# Autodesk Inventor assembly: Assembly1
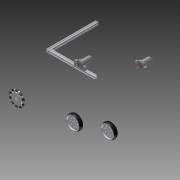
[picture p0: Inventor's stored thumbnail of the model, 180x180]
Saved by Autodesk Inventor 2013 (Build 170138000, 138)
## iProperties
Created: 2013-11-11
Part Number: Assembly1
Document SubType Name: Assembly
Designer: cobrooks
Author: cobrooks
## Documents named in this file (7)
- C:\Users\cobrooks\Documents\GitHub\2013-2014_BlockParty\CAD\Drive\WIMP_mk2\Assembly1.iam
- C:\Users\cobrooks\Documents\GitHub\2013-2014_BlockParty\CAD\COTSParts\Tetrix\Tetrix wheel 4 in.ipt
- C:\Users\cobrooks\Documents\GitHub\2013-2014_BlockParty\CAD\Drive\WIMP_mk2\DriveSide.ipt
- C:\Users\cobrooks\Documents\GitHub\2013-2014_BlockParty\CAD\COTSParts\Tetrix\Tetrix motor mount.ipt
- C:\Users\cobrooks\Documents\GitHub\2013-2014_BlockParty\CAD\Drive\WIMP_mk2\DriveBack.ipt
- C:\Users\cobrooks\Documents\GitHub\2013-2014_BlockParty\CAD\COTSParts\Tetrix\Tetrix motor.ipt
- C:\Users\cobrooks\Documents\GitHub\2013-2014_BlockParty\CAD\Drive\Final Drive Complete\Tetrix Wheel 4 in omni.ipt
## Components (9 placed, 6 different names)
1. Tetrix wheel 4 in:1 — Flush:1, Mate:1
2. Tetrix wheel 4 in:3 — Flush:1, Mate:4
3. DriveSide:1 — Mate:4, Mate:5, Flush:2, Flush:3, Flush:4, Mate:6, Flush:5
4. Tetrix motor mount:1 — Insert:1
5. Tetrix motor mount:2 — Insert:2, Flush:4, Mate:6, Flush:5
6. DriveBack:1 — Mate:5, Flush:2, Flush:3
7. Tetrix motor:1 — Insert:1
8. Tetrix motor:2 — Insert:2
9. Tetrix Wheel 4 in omni:1
## Relationships (11: Flush 5, Mate 4, Insert 2)
- Flush:1: Tetrix wheel 4 in:1 ↔ Tetrix wheel 4 in:3
- Mate:1: Tetrix wheel 4 in:1
- Mate:4: Tetrix wheel 4 in:3 ↔ DriveSide:1
- Mate:5: DriveSide:1 ↔ DriveBack:1
- Flush:2: DriveSide:1 ↔ DriveBack:1
- Flush:3: DriveSide:1 ↔ DriveBack:1
- Insert:1: Tetrix motor mount:1 ↔ Tetrix motor:1
- Insert:2: Tetrix motor mount:2 ↔ Tetrix motor:2
- Flush:4: DriveSide:1 ↔ Tetrix motor mount:2
- Mate:6: DriveSide:1 ↔ Tetrix motor mount:2
- Flush:5 (63.5 mm): DriveSide:1 ↔ Tetrix motor mount:2
